# Autodesk Inventor assembly: ArmFixture
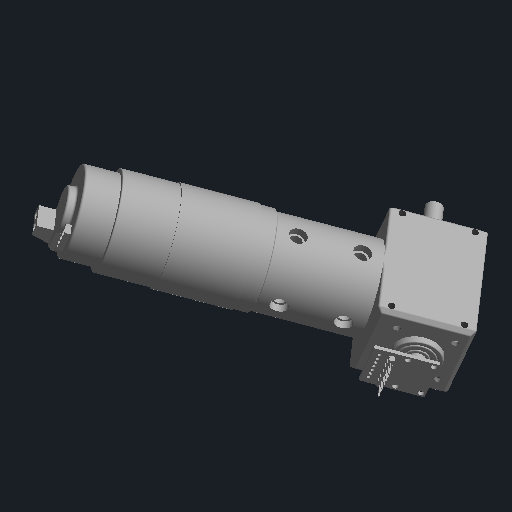
[picture p0: Inventor's stored thumbnail of the model, 512x512]
Saved by Autodesk Inventor 2025.2 (Build 292293000, 293)
## iProperties
Created: 2020-03-24
Part Number: ArmFixture
Document SubType Name: Assembly
Designer: valer
Mass: 715.256 g
Surface Area: 821.775 cm^2
Volume: 200.817 cm^3
Density: 3.56173 g/cm^3
Author: valer
## Documents named in this file (4)
- C:\Users\valer\Desktop\str1ker\cad\ArmFixture.iam
- C:\Users\valer\Desktop\str1ker\cad\external\ShoulderActuator\DumaDynamics00E.ipt
- C:\Users\valer\Desktop\str1ker\cad\external\ArmEncoder\ArmEncoderShaftMagnet6mm.ipt
- C:\Users\valer\Desktop\str1ker\cad\external\ShoulderEncoder\AS5040-AB-2.2-DemoBoard.ipt
## Components (3 placed, 3 different names)
1. DumaDynamics00E:1 — Flush:1, Mate:16, Mate:17, Flush:5, Mate:39, Angle:1
2. ArmEncoderShaftMagnet6mm:1 — Mate:16, Mate:17, Mate:42
3. AS5040-AB-2.2-DemoBoard:1 — Angle:1, Mate:42
## Relationships (7: Mate 4, Flush 2, Angle 1)
- Flush:1: DumaDynamics00E:1
- Mate:16: DumaDynamics00E:1 ↔ ArmEncoderShaftMagnet6mm:1
- Mate:17: DumaDynamics00E:1 ↔ ArmEncoderShaftMagnet6mm:1
- Flush:5 (6 mm): DumaDynamics00E:1
- Mate:39: DumaDynamics00E:1
- Angle:1 (0 deg): DumaDynamics00E:1 ↔ AS5040-AB-2.2-DemoBoard:1
- Mate:42 (0.15 mm): ArmEncoderShaftMagnet6mm:1 ↔ AS5040-AB-2.2-DemoBoard:1
